# Autodesk Inventor assembly: cRIO-FRC PCB
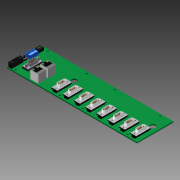
[picture p0: Inventor's stored thumbnail of the model, 180x180]
Saved by Autodesk Inventor 2011 (Build 150239000, 239)
## iProperties
Category: FIRST
Manager: Ed Sparks
Company: FirstCadLibrary
Shininess: 64.0
Length Units: 11272
Angle Units: 11279
Time Units: 11290
Mass Units: 11286
Length Display Precision: 3
Angle Display Precision: 2
Compacted: True
Part Number: cRIO-FRC PCB
Document SubType Name: Assembly
Created: 2008-12-13
Designer: Ed Sparks
Project: FIRST
Catalog Web Link: www.firstcadlibrary.com
Engineer: Ed Sparks
Density: 0.0
Volumn: 0.0
Area: 0.0
PropertySet Name: Model Information
Control State: 0
Master: False
Checked Out: False
Author: Ed Sparks
Keywords: FIRST
## Documents named in this file (9)
- R:\CAD Archives\Electronics\cRIO 1764\cRIO PCB 1764.iam
- R:\CAD Archives\Electronics\cRIO 1764\cRIO Electric board 1764.ipt
- R:\CAD Archives\Electronics\cRIO 1764\cRIO LED 1764.ipt
- R:\CAD Archives\Electronics\cRIO 1764\Power Connector 1764.ipt
- R:\CAD Archives\Electronics\cRIO 1764\DIP Switch 1764.ipt
- R:\CAD Archives\Electronics\cRIO 1764\DB-15HDM 1764.ipt
- R:\CAD Archives\Electronics\cRIO 1764\cRIO Switch 1764.ipt
- R:\CAD Archives\Electronics\cRIO 1764\9M D-Shell 1764.ipt
- R:\CAD Archives\Electronics\cRIO 1764\CAT5 1764.ipt
## Components (16 placed, 8 different names)
1. cRIO Electric Board 1764:1 — Mate:1, Flush:1, Flush:2, Mate:2, Flush:3, Flush:4, Mate:3, Flush:5, Flush:6, Mate:4, Flush:7, Flush:8, Mate:5, Flush:9, 1.51, Mate:6, Flush:10, Flush:11, Mate:7, Flush:12, Flush:13
2. cRIO LED 1764:1 — Mate:1, Flush:1, Flush:2
3. Power Connector 1764:1 — Mate:2, Flush:3, Flush:4
4. cRIO Switch 1764:1 — Mate:3, Flush:5, Flush:6
5. 9M D-Shell 1764:1 — Mate:4, Flush:7, Flush:8
6. DIP Switch 1764:1 — Mate:5, Flush:9, 1.51
7. DB-15HDM 1764:1 — Mate:6, Flush:10, Flush:11
8. DB-15HDM 1764:2
9. DB-15HDM 1764:3
10. DB-15HDM 1764:4
11. DB-15HDM 1764:5
12. DB-15HDM 1764:6
13. DB-15HDM 1764:7
14. DB-15HDM 1764:8
15. CAT5 1764:1 — Mate:7, Flush:12, Flush:13
16. CAT5 1764:2
## Component patterns: (8 elements, first: DB-15HDM 1764:1), (2 elements, first: CAT5 1764:1)
## Relationships (21: Flush 14, Mate 7)
- Mate:1: cRIO Electric Board 1764:1 ↔ cRIO LED 1764:1
- Flush:1 (7.366 mm): cRIO Electric Board 1764:1 ↔ cRIO LED 1764:1
- Flush:2 (-1.016 mm): cRIO Electric Board 1764:1 ↔ cRIO LED 1764:1
- Mate:2: cRIO Electric Board 1764:1 ↔ Power Connector 1764:1
- Flush:3 (1.1176 mm): cRIO Electric Board 1764:1 ↔ Power Connector 1764:1
- Flush:4 (1.651 mm): cRIO Electric Board 1764:1 ↔ Power Connector 1764:1
- Mate:3: cRIO Electric Board 1764:1 ↔ cRIO Switch 1764:1
- Flush:5 (-28.575 mm): cRIO Electric Board 1764:1 ↔ cRIO Switch 1764:1
- Flush:6 (1.524 mm): cRIO Electric Board 1764:1 ↔ cRIO Switch 1764:1
- Mate:4: cRIO Electric Board 1764:1 ↔ 9M D-Shell 1764:1
- Flush:7 (17.78 mm): cRIO Electric Board 1764:1 ↔ 9M D-Shell 1764:1
- Flush:8 (13.97 mm): cRIO Electric Board 1764:1 ↔ 9M D-Shell 1764:1
- Mate:5: cRIO Electric Board 1764:1 ↔ DIP Switch 1764:1
- Flush:9 (0.889 mm): cRIO Electric Board 1764:1 ↔ DIP Switch 1764:1
- 1.51 [Flush] (38.354 mm): cRIO Electric Board 1764:1 ↔ DIP Switch 1764:1
- Mate:6: cRIO Electric Board 1764:1 ↔ DB-15HDM 1764:1
- Flush:10 (4.064 mm): cRIO Electric Board 1764:1 ↔ DB-15HDM 1764:1
- Flush:11 (5.842 mm): cRIO Electric Board 1764:1 ↔ DB-15HDM 1764:1
- Mate:7: cRIO Electric Board 1764:1 ↔ CAT5 1764:1
- Flush:12 (2.794 mm): cRIO Electric Board 1764:1 ↔ CAT5 1764:1
- Flush:13 (46.482 mm): cRIO Electric Board 1764:1 ↔ CAT5 1764:1
